# Autodesk Inventor assembly: Test_assembly
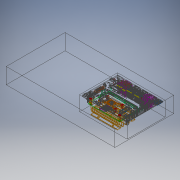
[picture p0: Inventor's stored thumbnail of the model, 180x180]
Saved by Autodesk Inventor 2019 (Build 230136000, 136)
## iProperties
Created: 2020-02-14
Part Number: Test_assembly
Document SubType Name: Assembly
Designer: close
Author: close
## Documents named in this file (3)
- C:\Users\close\Desktop\CAD BARC-ROAR\Enclosure\V_2\Test_assembly.iam
- C:\Users\close\Desktop\CAD BARC-ROAR\Enclosure\V_2\Enclosure_v2.ipt
- C:\Users\close\Desktop\CAD BARC-ROAR\Dependencies\Nvidia Jetson Nano\P3450_P3449_A02_P3448_A02.iam
## Components (2 placed, 2 different names)
1. Enclosure_v2:1 — Insert:1, Insert:2
2. P3450_P3449_A02_P3448_A02:1 [sub-assembly] — Insert:1, Insert:2
## Relationships (2: Insert 2)
- Insert:1: Enclosure_v2:1 ↔ P3450_P3449_A02_P3448_A02:1
- Insert:2: Enclosure_v2:1 ↔ P3450_P3449_A02_P3448_A02:1
